# Autodesk Inventor assembly: hc-sr04_servo_mount
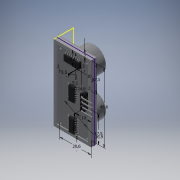
[picture p0: Inventor's stored thumbnail of the model, 180x180]
Saved by Autodesk Inventor 2019 (Build 230136000, 136)
## iProperties
Created: 2018-08-20
Part Number: hc-sr04_servo_mount
Document SubType Name: Assembly
Designer: ndz
Author: ndz
## Documents named in this file (3)
- E:\Dropbox\_PRACA\HARDWARE\IE-TRACK-KIT-PWR-1\hc-sr04_servo_mount.iam
- E:\Dropbox\_PRACA\HARDWARE\IE-TRACK-KIT-PWR-1\MECH\v12\hc-sr04_servo_mount.ipt
- E:\Dropbox\_PRACA\HARDWARE\IE-TRACK-KIT-PWR-1\MECH\v12\HC-SR04-UltrasonicSensor v7.ipt
## Components (2 placed, 2 different names)
1. hc-sr04_servo_mount:1 — Mate:1, Mate:2, Mate:3, Mate:4, Mate:5
2. HC-SR04-UltrasonicSensor v7:1 — Mate:3, Mate:4, Mate:5
## Relationships (5: Mate 5)
- Mate:1: hc-sr04_servo_mount:1
- Mate:2: hc-sr04_servo_mount:1
- Mate:3: hc-sr04_servo_mount:1 ↔ HC-SR04-UltrasonicSensor v7:1
- Mate:4: hc-sr04_servo_mount:1 ↔ HC-SR04-UltrasonicSensor v7:1
- Mate:5: hc-sr04_servo_mount:1 ↔ HC-SR04-UltrasonicSensor v7:1
